# Autodesk Inventor assembly: estação_bga_3
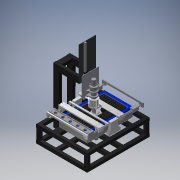
[picture p0: Inventor's stored thumbnail of the model, 180x180]
Saved by Autodesk Inventor 2018 (Build 220112000, 112)
## iProperties
Created: 2018-07-20
Part Number: estação_bga_3
Material: Genérico
Document SubType Name: Assembly
Designer: Usuario
Mass: 28977.3 g
Surface Area: 37496.8 cm^2
Volume: 6730.78 cm^3
Density: 4.30519 g/cm^3
Author: Usuario
## Documents named in this file (8)
- C:\Users\Usuario\Desktop\Estação BGA\Peças 3D\estação_bga_3.iam
- C:\Users\Usuario\Desktop\Estação BGA\Peças 3D\mesa_aquecimento_fresamento.iam
- C:\Users\Usuario\Desktop\Estação BGA\Peças 3D\estrutura.iam
- C:\Users\Usuario\Desktop\Estação BGA\Peças 3D\mesa_suporte_de_placa.iam
- C:\Users\Usuario\Desktop\Estação BGA\Peças 3D\cabeça_inferior.iam
- C:\Users\Usuario\Desktop\Estação BGA\Peças 3D\bocal_inferior.ipt
- C:\Users\Usuario\Desktop\Estação BGA\Peças 3D\ApoioBocalInferior_.ipt
- C:\Users\Usuario\Desktop\Estação BGA\Peças 3D\cabeça_superior_4.iam
## Components (7 placed, 7 different names)
1. mesa_aquecimento_fresamento:1 [sub-assembly] — Coincidência:11, Coincidência:14, Ângulo:1, Coincidência:15, Alinhamento:6, Coincidência:16
2. estrutura:1 [sub-assembly] — Coincidência:6, Alinhamento:2, Coincidência:8, Coincidência:14, Coincidência:17, Alinhamento:7, Alinhamento:8, Coincidência:18
3. mesa_suporte_de_placa:1 [sub-assembly] — Coincidência:15, Alinhamento:6, Coincidência:16
4. cabeça_inferior:1 [sub-assembly] — Coincidência:7, Alinhamento:3, Coincidência:9, Coincidência:10, Alinhamento:4, Coincidência:11
5. bocal_inferior:1 — Coincidência:9, Coincidência:10
6. ApoioBocalInferior_:1 — Coincidência:6, Alinhamento:2, Coincidência:7, Alinhamento:3, Coincidência:8, Alinhamento:4, Ângulo:1
7. cabeça_superior_4:1 [sub-assembly] — Coincidência:17, Alinhamento:7, Alinhamento:8
## Relationships (18: Mate 11, Flush 6, Angle 1)
- Coincidência:6 [Mate]: estrutura:1 ↔ ApoioBocalInferior_:1
- Alinhamento:2 [Flush]: estrutura:1 ↔ ApoioBocalInferior_:1
- Coincidência:7 [Mate]: cabeça_inferior:1 ↔ ApoioBocalInferior_:1
- Alinhamento:3 [Flush] (28 mm): cabeça_inferior:1 ↔ ApoioBocalInferior_:1
- Coincidência:8 [Mate]: estrutura:1 ↔ ApoioBocalInferior_:1
- Coincidência:9 [Mate]: cabeça_inferior:1 ↔ bocal_inferior:1
- Coincidência:10 [Mate]: cabeça_inferior:1 ↔ bocal_inferior:1
- Alinhamento:4 [Flush] (45 mm): cabeça_inferior:1 ↔ ApoioBocalInferior_:1
- Coincidência:11 [Mate]: mesa_aquecimento_fresamento:1 ↔ cabeça_inferior:1
- Coincidência:14 [Mate]: mesa_aquecimento_fresamento:1 ↔ estrutura:1
- Ângulo:1 [Angle] (90 deg): mesa_aquecimento_fresamento:1 ↔ ApoioBocalInferior_:1
- Coincidência:15 [Mate] (17.016 mm): mesa_aquecimento_fresamento:1 ↔ mesa_suporte_de_placa:1
- Alinhamento:6 [Flush]: mesa_aquecimento_fresamento:1 ↔ mesa_suporte_de_placa:1
- Coincidência:16 [Mate] (40.48 mm): mesa_aquecimento_fresamento:1 ↔ mesa_suporte_de_placa:1
- Coincidência:17 [Mate]: estrutura:1 ↔ cabeça_superior_4:1
- Alinhamento:7 [Flush]: estrutura:1 ↔ cabeça_superior_4:1
- Alinhamento:8 [Flush]: estrutura:1 ↔ cabeça_superior_4:1
- Coincidência:18 [Mate]: estrutura:1
## Named parameters: sa_0 = -1.2153e-09, sa_1 = -2.98637e-07, sa_2 = -1000
note: some values were not read from the file. Shown as the stored number, unit unknown: "sa_0", "sa_1", "sa_2".
